# Autodesk Inventor assembly: leg_motor_moudle_MIR
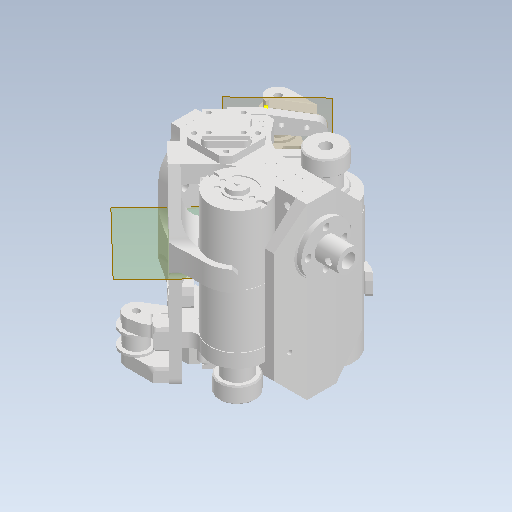
[picture p0: Inventor's stored thumbnail of the model, 512x512]
Saved by Autodesk Inventor 2020 (Build 240168000, 168)
## iProperties
Created: 2019-05-09
Part Number: leg_motor_moudle_MIR
Document SubType Name: Assembly
Designer: psrob
Author: psrob
## Documents named in this file (18)
- E:\projects-2\project dog gen2\hardware\leg_motor_moudle_MIR.iam
- E:\projects-2\project dog gen2\hardware\leg_basket_1_MIR.ipt
- E:\projects-2\project dog gen2\hardware\leg_basket_2_MIR.ipt
- E:\projects-2\project dog gen2\hardware\motor_holder_MIR.ipt
- E:\projects-2\project dog gen2\hardware\leg_basket_3_MIR.ipt
- E:\projects-2\project dog gen2\hardware\pin_3_14_MIR.ipt
- E:\projects-2\project dog gen2\hardware\motor_2_MIR.ipt
- E:\projects-2\project dog gen2\hardware\pin_6_20_MIR.ipt
- E:\projects-2\project dog gen2\hardware\pin_6_60_MIR.ipt
- E:\projects-2\project dog gen2\hardware\2GT_wheel_MIR.ipt
- E:\projects-2\project dog gen2\hardware\bearing_6_13_5_MIR.ipt
- E:\projects-2\project dog gen2\hardware\flange_6mm_MIR.ipt
- E:\projects-2\project dog gen2\hardware\cross_axis_holder_1_MIR.ipt
- E:\projects-2\project dog gen2\hardware\2GT_wheel_5_MIR.ipt
- E:\projects-2\project dog gen2\hardware\encoder_ass_MIR.iam
- E:\projects-2\project dog gen2\hardware\wheel_holder_2_MIR.ipt
- E:\projects-2\project dog gen2\hardware\wheel_holder_1_MIR.ipt
- E:\projects-2\project dog gen2\hardware\2GT_wheel1_MIR.ipt
## Components (31 placed, 17 different names)
1. leg_basket_1_MIR:1 — Insert:6, Insert:5, Insert:8, Insert:7, Insert:2, Insert:1, Insert:4, Insert:3, Insert:29, Insert:28
2. leg_basket_2_MIR:1 — Insert:6, Insert:5, Insert:12, Insert:9, Insert:15, Insert:24, Insert:26, Insert:34, Insert:35
3. leg_basket_2_MIR:2 — Insert:8, Insert:7, Insert:11, Insert:10, Insert:14, Insert:25, Tangent:2, Mate:1, Insert:27, Insert:32, Insert:33
4. motor_holder_MIR:1 — Insert:2, Insert:1, Insert:16, Insert:20, Insert:19
5. motor_holder_MIR:2 — Insert:4, Insert:3, Insert:13, Insert:18, Insert:17
6. leg_basket_3_MIR:1 — Insert:12, Insert:11, Flush:1, Insert:40, Insert:41, Mate:4
7. leg_basket_3_MIR:2 — Insert:10, Insert:9, Insert:36, Insert:37, Mate:3
8. pin_3_14_MIR:1 — Insert:13
9. pin_3_14_MIR:2 — Insert:14
10. pin_3_14_MIR:3 — Insert:16
11. pin_3_14_MIR:4 — Insert:15
12. motor_2_MIR:1 — Insert:20, Insert:19, Insert:30
13. motor_2_MIR:2 — Insert:18, Insert:17, Insert:31
14. pin_6_20_MIR:1 — Insert:22
15. pin_6_60_MIR:1 — Insert:21, Insert:23, Tangent:1
16. 2GT_wheel_MIR:1 — Insert:21
17. bearing_6_13_5_MIR:1 — Insert:24, Insert:22
18. bearing_6_13_5_MIR:2 — Insert:25, Insert:23
19. flange_6mm_MIR:1 — Tangent:2, Tangent:1, Mate:1
20. cross_axis_holder_1_MIR:1 — Flush:1, Insert:27, Insert:26
21. flange_6mm_MIR:2 — Insert:29, Insert:28
22. 2GT_wheel_5_MIR:1 — Insert:31
23. 2GT_wheel_5_MIR:2 — Insert:30
24. encoder_ass_MIR:1 [sub-assembly] — Insert:32, Insert:33
25. encoder_ass_MIR:2 [sub-assembly] — Insert:34, Insert:35
26. wheel_holder_2_MIR:1 — Insert:39, Mate:3
27. wheel_holder_1_MIR:1 — Insert:36, Insert:37, Insert:38
28. 2GT_wheel1_MIR:1 — Insert:38, Insert:39
29. wheel_holder_2_MIR:2 — Insert:43, Mate:4
30. wheel_holder_1_MIR:2 — Insert:40, Insert:41, Insert:42
31. 2GT_wheel1_MIR:2 — Insert:42, Insert:43
## Relationships (49: Insert 43, Mate 4, Tangent 2)
- Insert:6: leg_basket_1_MIR:1 ↔ leg_basket_2_MIR:1
- Insert:5: leg_basket_1_MIR:1 ↔ leg_basket_2_MIR:1
- Insert:8: leg_basket_1_MIR:1 ↔ leg_basket_2_MIR:2
- Insert:7: leg_basket_1_MIR:1 ↔ leg_basket_2_MIR:2
- Insert:2: leg_basket_1_MIR:1 ↔ motor_holder_MIR:1
- Insert:1: leg_basket_1_MIR:1 ↔ motor_holder_MIR:1
- Insert:4: leg_basket_1_MIR:1 ↔ motor_holder_MIR:2
- Insert:3: leg_basket_1_MIR:1 ↔ motor_holder_MIR:2
- Insert:12: leg_basket_2_MIR:1 ↔ leg_basket_3_MIR:1
- Insert:11: leg_basket_2_MIR:2 ↔ leg_basket_3_MIR:1
- Insert:10: leg_basket_2_MIR:2 ↔ leg_basket_3_MIR:2
- Insert:9: leg_basket_2_MIR:1 ↔ leg_basket_3_MIR:2
- Insert:13: motor_holder_MIR:2 ↔ pin_3_14_MIR:1
- Insert:14: leg_basket_2_MIR:2 ↔ pin_3_14_MIR:2
- Insert:16: motor_holder_MIR:1 ↔ pin_3_14_MIR:3
- Insert:15: leg_basket_2_MIR:1 ↔ pin_3_14_MIR:4
- Insert:20: motor_holder_MIR:1 ↔ motor_2_MIR:1
- Insert:19: motor_holder_MIR:1 ↔ motor_2_MIR:1
- Insert:18: motor_holder_MIR:2 ↔ motor_2_MIR:2
- Insert:17: motor_holder_MIR:2 ↔ motor_2_MIR:2
- Insert:21 (-21 mm): pin_6_60_MIR:1 ↔ 2GT_wheel_MIR:1
- Insert:24: leg_basket_2_MIR:1 ↔ bearing_6_13_5_MIR:1
- Insert:22: pin_6_20_MIR:1 ↔ bearing_6_13_5_MIR:1
- Insert:25: leg_basket_2_MIR:2 ↔ bearing_6_13_5_MIR:2
- Insert:23: pin_6_60_MIR:1 ↔ bearing_6_13_5_MIR:2
- Tangent:2: leg_basket_2_MIR:2 ↔ flange_6mm_MIR:1
- Tangent:1: pin_6_60_MIR:1 ↔ flange_6mm_MIR:1
- Mate:1 (-5 mm): leg_basket_2_MIR:2 ↔ flange_6mm_MIR:1
- Flush:1 [Mate]: leg_basket_3_MIR:1 ↔ cross_axis_holder_1_MIR:1
- Insert:27: leg_basket_2_MIR:2 ↔ cross_axis_holder_1_MIR:1
- Insert:26: leg_basket_2_MIR:1 ↔ cross_axis_holder_1_MIR:1
- Insert:29: leg_basket_1_MIR:1 ↔ flange_6mm_MIR:2
- Insert:28: leg_basket_1_MIR:1 ↔ flange_6mm_MIR:2
- Insert:31 (-3 mm): motor_2_MIR:2 ↔ 2GT_wheel_5_MIR:1
- Insert:30 (-3 mm): motor_2_MIR:1 ↔ 2GT_wheel_5_MIR:2
- Insert:32: leg_basket_2_MIR:2 ↔ encoder_ass_MIR:1
- Insert:33: leg_basket_2_MIR:2 ↔ encoder_ass_MIR:1
- Insert:34: leg_basket_2_MIR:1 ↔ encoder_ass_MIR:2
- Insert:35: leg_basket_2_MIR:1 ↔ encoder_ass_MIR:2
- Insert:36: leg_basket_3_MIR:2 ↔ wheel_holder_1_MIR:1
- Insert:37: leg_basket_3_MIR:2 ↔ wheel_holder_1_MIR:1
- Insert:38: wheel_holder_1_MIR:1 ↔ 2GT_wheel1_MIR:1
- Insert:39: wheel_holder_2_MIR:1 ↔ 2GT_wheel1_MIR:1
- Mate:3: leg_basket_3_MIR:2 ↔ wheel_holder_2_MIR:1
- Insert:40: leg_basket_3_MIR:1 ↔ wheel_holder_1_MIR:2
- Insert:41: leg_basket_3_MIR:1 ↔ wheel_holder_1_MIR:2
- Insert:42: wheel_holder_1_MIR:2 ↔ 2GT_wheel1_MIR:2
- Insert:43: wheel_holder_2_MIR:2 ↔ 2GT_wheel1_MIR:2
- Mate:4: leg_basket_3_MIR:1 ↔ wheel_holder_2_MIR:2
